# Autodesk Inventor assembly: LegEnd_MIR
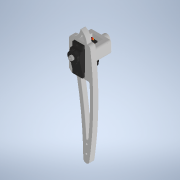
[picture p0: Inventor's stored thumbnail of the model, 180x180]
Saved by Autodesk Inventor 2020.3 (Build 243373000, 373)
## iProperties
Created: 2022-03-31
Part Number: LegEnd_MIR
Document SubType Name: Assembly
Designer: sanyi
Author: sanyi
## Documents named in this file (4)
- C:\Users\sanyi\OneDrive\Dokumentumok\Inventor\Quadropod\Quadropod MDL\AssemblyForSimulationModell\LegEnd_MIR.iam
- C:\Users\sanyi\OneDrive\Dokumentumok\Inventor\Quadropod\LegEnd_Right_v2_MIR.ipt
- C:\Users\sanyi\OneDrive\Dokumentumok\Inventor\Quadropod\LegPin_v1.ipt
- C:\Users\sanyi\OneDrive\Dokumentumok\Inventor\Quadropod\SH-0257MG.ipt
## Components (3 placed, 3 different names)
1. LegEnd_Right_v2_MIR:1 — Insert:1, Insert:2, Insert:3, Angle:1
2. LegPin_v1:1 — Insert:1, Insert:2
3. SH-0257MG:1 — Insert:3, Angle:1
## Relationships (4: Insert 3, Angle 1)
- Insert:1: LegEnd_Right_v2_MIR:1 ↔ LegPin_v1:1
- Insert:2: LegEnd_Right_v2_MIR:1 ↔ LegPin_v1:1
- Insert:3: LegEnd_Right_v2_MIR:1 ↔ SH-0257MG:1
- Angle:1 (180 deg): LegEnd_Right_v2_MIR:1 ↔ SH-0257MG:1
